# Autodesk Inventor assembly: 3DPrinter
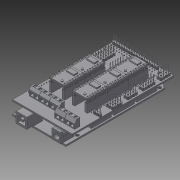
[picture p0: Inventor's stored thumbnail of the model, 180x180]
Saved by Autodesk Inventor 2014 (Build 180170000, 170)
## iProperties
Created: 2014-11-11
Part Number: 3DPrinter
Document SubType Name: Assembly
Designer: ThatOtherGuy
Author: ThatOtherGuy
## Documents named in this file (3)
- C:\Users\ThatOtherGuy\Documents\Inventor\KosselCNC1515\Electronics\3DPrinter.iam
- C:\Users\ThatOtherGuy\Documents\Inventor\KosselCNC1515\Electronics\Arduino_Mega2560_R3.iam
- C:\Users\ThatOtherGuy\Documents\Inventor\KosselCNC1515\Electronics\RAMPS14.iam
## Components (2 placed, 2 different names)
1. Arduino_Mega2560_R3:1 [sub-assembly] — Insert:1, Insert:2
2. RAMPS14:1 [sub-assembly] — Insert:1, Insert:2
## Relationships (2: Insert 2)
- Insert:1 (0.5 mm): Arduino_Mega2560_R3:1 ↔ RAMPS14:1
- Insert:2 (0.5 mm): Arduino_Mega2560_R3:1 ↔ RAMPS14:1
